# Autodesk Inventor assembly: Ground_Tracker
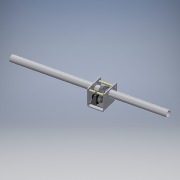
[picture p0: Inventor's stored thumbnail of the model, 180x180]
Saved by Autodesk Inventor 2018 (Build 220112000, 112)
## iProperties
Created: 2018-09-27
Part Number: Ground_Tracker
Document SubType Name: Assembly
Designer: Bradley
Author: Bradley
## Documents named in this file (11)
- C:\Users\Bradley\Documents\GitHub\CougSat1-Hardware\CougSat1-GroundStation\CADModel\Native\Ground_Tracker.iam
- C:\Users\Bradley\Documents\GitHub\CougSat1-Hardware\CougSat1-GroundStation\CADModel\Native\Ground_Tracker_TripodMount.ipt
- C:\Users\Bradley\Documents\GitHub\CougSat1-Hardware\CougSat1-GroundStation\CADModel\Native\Ground_Tracker_Bearing.ipt
- C:\Users\Bradley\Documents\GitHub\CougSat1-Hardware\CougSat1-GroundStation\CADModel\Native\Ground_Tracker_CrossTube.ipt
- C:\Users\Bradley\Documents\GitHub\Resources\ComponentModels\Hardware\Coupler_ServoHub.ipt
- C:\Users\Bradley\Documents\GitHub\Resources\ComponentModels\Electronics\Servo_Standard.ipt
- C:\Users\Bradley\Documents\GitHub\CougSat1-Hardware\CougSat1-GroundStation\CADModel\Native\Ground_Tracker_Spacer.ipt
- C:\Users\Bradley\Documents\GitHub\CougSat1-Hardware\CougSat1-GroundStation\CADModel\Native\Ground_Tracker_ServoMount.ipt
- C:\Users\Bradley\Documents\GitHub\CougSat1-Hardware\CougSat1-GroundStation\CADModel\Native\Ground_Tracker_ElevationGear.ipt
- C:\Users\Bradley\Documents\GitHub\CougSat1-Hardware\CougSat1-GroundStation\CADModel\Native\Ground_Tracker_ElevationPinion.ipt
- C:\Users\Bradley\Documents\GitHub\CougSat1-Hardware\CougSat1-GroundStation\CADModel\Native\Ground_Tracker_CrossTubeCollar.ipt
## Components (14 placed, 10 different names)
1. Ground_Tracker_TripodMount:1 — Insert:1, Insert:8, Insert:9
2. Ground_Tracker_Bearing:1 — Insert:1, Mate:1, Flush:1, Insert:5, Insert:6, Insert:12, Insert:13, Insert:18, Insert:19
3. Ground_Tracker_CrossTube:1 — Mate:1, Flush:1, Mate:2
4. Coupler_ServoHub:1 — Insert:4, Insert:8, Insert:9
5. Servo_Standard:1 — Insert:4, Insert:10, Insert:11
6. Servo_Standard:2 — Insert:7, Insert:14, Insert:15
7. Ground_Tracker_Spacer:1 — Insert:5
8. Ground_Tracker_Spacer:2 — Insert:6, Mate:3
9. Coupler_ServoHub:2 — Insert:7, Insert:16, Insert:17
10. Ground_Tracker_ServoMount:1 — Insert:10, Insert:11, Insert:12, Insert:13, Insert:14, Insert:15, Mate:3
11. Ground_Tracker_ElevationGear:1 — Flush:2, Mate:2
12. Ground_Tracker_ElevationPinion:1 — Insert:16, Insert:17, Flush:2
13. Ground_Tracker_CrossTubeCollar:1 — Insert:18
14. Ground_Tracker_CrossTubeCollar:2 — Insert:19
## Relationships (22: Insert 17, Mate 3, Flush 2)
- Insert:1: Ground_Tracker_TripodMount:1 ↔ Ground_Tracker_Bearing:1
- Mate:1: Ground_Tracker_Bearing:1 ↔ Ground_Tracker_CrossTube:1
- Flush:1 (70 mm): Ground_Tracker_Bearing:1 ↔ Ground_Tracker_CrossTube:1
- Insert:4: Coupler_ServoHub:1 ↔ Servo_Standard:1
- Insert:5: Ground_Tracker_Bearing:1 ↔ Ground_Tracker_Spacer:1
- Insert:6: Ground_Tracker_Bearing:1 ↔ Ground_Tracker_Spacer:2
- Insert:7: Servo_Standard:2 ↔ Coupler_ServoHub:2
- Insert:8: Ground_Tracker_TripodMount:1 ↔ Coupler_ServoHub:1
- Insert:9: Ground_Tracker_TripodMount:1 ↔ Coupler_ServoHub:1
- Insert:10: Servo_Standard:1 ↔ Ground_Tracker_ServoMount:1
- Insert:11: Servo_Standard:1 ↔ Ground_Tracker_ServoMount:1
- Insert:12: Ground_Tracker_Bearing:1 ↔ Ground_Tracker_ServoMount:1
- Insert:13: Ground_Tracker_Bearing:1 ↔ Ground_Tracker_ServoMount:1
- Insert:14: Servo_Standard:2 ↔ Ground_Tracker_ServoMount:1
- Insert:15: Servo_Standard:2 ↔ Ground_Tracker_ServoMount:1
- Insert:16: Coupler_ServoHub:2 ↔ Ground_Tracker_ElevationPinion:1
- Insert:17: Coupler_ServoHub:2 ↔ Ground_Tracker_ElevationPinion:1
- Flush:2: Ground_Tracker_ElevationGear:1 ↔ Ground_Tracker_ElevationPinion:1
- Mate:2: Ground_Tracker_CrossTube:1 ↔ Ground_Tracker_ElevationGear:1
- Mate:3: Ground_Tracker_Spacer:2 ↔ Ground_Tracker_ServoMount:1
- Insert:18: Ground_Tracker_Bearing:1 ↔ Ground_Tracker_CrossTubeCollar:1
- Insert:19: Ground_Tracker_Bearing:1 ↔ Ground_Tracker_CrossTubeCollar:2
